# Autodesk Inventor assembly: !tower
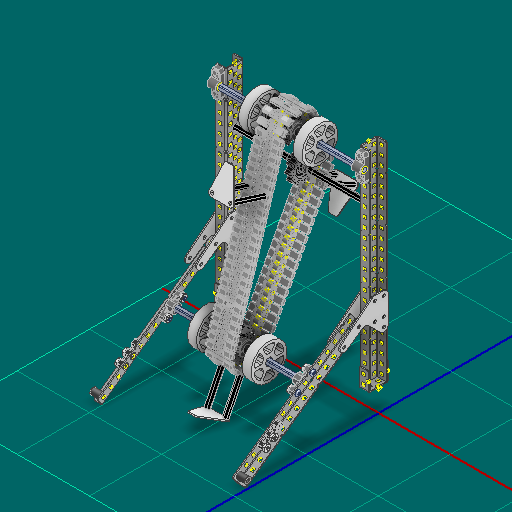
[picture p0: Inventor's stored thumbnail of the model, 512x512]
Saved by Autodesk Inventor 2025 (Build 290162000, 162)
## iProperties
Created: 2024-10-13
Part Number: !tower
Document SubType Name: Assembly
Designer: Averey Ku
Author: Averey Ku
## Documents named in this file (26)
- C:\Users\avere\vex_robotics_high_stakes\hardware\cad\bots\high_stakes_v2\tower\!tower.iam
- C:\Users\avere\vex_robotics_high_stakes\hardware\cad\bots\high_stakes_v2\tower\structure\!structure.iam
- C:\Users\avere\vex_robotics_high_stakes\hardware\cad\robpros_cad_lib\Motion\Shaft HS\Shaft HS\Shaft HS 7.5 in.ipt
- C:\Users\avere\vex_robotics_high_stakes\hardware\cad\robpros_cad_lib\Motion\Sprockets\9P Sprocket\9P 12T Sprocket, No Insert.iam
- C:\Users\avere\vex_robotics_high_stakes\hardware\cad\robpros_cad_lib\Motion\Wheels\Flex Wheels\2.000 Flex Wheel\2.000 30A .500.ipt
- C:\Users\avere\vex_robotics_high_stakes\hardware\cad\robpros_cad_lib\Motion\Shaft HS\Shaft HS\Shaft HS 8.5 in.ipt
- C:\Users\avere\vex_robotics_high_stakes\hardware\cad\bots\high_stakes_v2\tower\chain_path.ipt
- C:\Users\avere\vex_robotics_high_stakes\hardware\cad\robpros_cad_lib\Motion\Chain 9P\Tank Tread Traction Link.ipt
- C:\Users\avere\vex_robotics_high_stakes\hardware\cad\robpros_cad_lib\Motion\Chain 9P\Chain Attachment Link.ipt
- C:\Users\avere\vex_robotics_high_stakes\hardware\cad\robpros_cad_lib\Structure\Standoff\Standoff .25.ipt
- C:\Users\avere\vex_robotics_high_stakes\hardware\cad\robpros_cad_lib\Structure\Standoff\Standoff 3.00.ipt
- C:\Users\avere\vex_robotics_high_stakes\hardware\cad\robpros_cad_lib\Motion\Spacers\Spacer Nylon .375 OD\NSpacer .375 OD x .125.ipt
- C:\Users\avere\vex_robotics_high_stakes\hardware\cad\robpros_cad_lib\Motion\Spacers\Washer Steel\SWasher .375 OD x .031250.ipt
- C:\Users\avere\vex_robotics_high_stakes\hardware\cad\robpros_cad_lib\Structure\Standoff\Standoff 2.00.ipt
- C:\Users\avere\vex_robotics_high_stakes\hardware\cad\bots\high_stakes_v2\intake\custom_parts\hook_gusset.ipt
- C:\Users\avere\vex_robotics_high_stakes\hardware\cad\robpros_cad_lib\Motion\Shaft HS\HS Spacer\HSpacer .0625.ipt
- C:\Users\avere\vex_robotics_high_stakes\hardware\cad\robpros_cad_lib\Motion\Shaft HS\HS Spacer.ipt
- C:\Users\avere\vex_robotics_high_stakes\hardware\cad\robpros_cad_lib\Motion\Shaft HS\HS Spacer\HSpacer .1250.ipt
- C:\Users\avere\vex_robotics_high_stakes\hardware\cad\robpros_cad_lib\Motion\Shaft HS\HS Spacer\HSpacer .5000.ipt
- C:\Users\avere\vex_robotics_high_stakes\hardware\cad\robpros_cad_lib\Motion\Shaft HS\Low Profile HS Shaft Collar.ipt
- C:\Users\avere\vex_robotics_high_stakes\hardware\cad\robpros_cad_lib\Motion\Shaft HS\Shaft HS.ipt
- C:\Users\avere\vex_robotics_high_stakes\hardware\cad\robpros_cad_lib\Motion\Sprockets\9P Sprocket.iam
- C:\Users\avere\vex_robotics_high_stakes\hardware\cad\robpros_cad_lib\Motion\Wheels\Flex Wheels\2.000 Flex Wheel.ipt
- C:\Users\avere\vex_robotics_high_stakes\hardware\cad\robpros_cad_lib\Structure\Standoff.ipt
- C:\Users\avere\vex_robotics_high_stakes\hardware\cad\robpros_cad_lib\Motion\Spacers\Spacer Nylon .375 OD.ipt
- C:\Users\avere\vex_robotics_high_stakes\hardware\cad\robpros_cad_lib\Motion\Spacers\Washer Steel.ipt
## Components (111 placed, 18 different names)
1. !structure:1 [sub-assembly] — Insert:1, Insert:2, Insert:5, Insert:11, Insert:17
2. Shaft HS 7.5 in:1 — Insert:1
3. 9P 12T Sprocket, No Insert:2 [sub-assembly] — Insert:2, Insert:3, Insert:4, Flush:1, Flush:3, Insert:41, Insert:42
4. 2.000 30A .500:1 — Insert:3
5. 2.000 30A .500:2 — Insert:4
6. Shaft HS 8.5 in:2 — Insert:5, Mate:1
7. 9P 12T Sprocket, No Insert:3 [sub-assembly] — Flush:1, Mate:1, Insert:6, Insert:7, Flush:2, Mate:3, Insert:49, Insert:50
8. 2.000 30A .500:3 — Insert:6
9. 2.000 30A .500:4 — Insert:7
10. 9P 12T Sprocket, No Insert:4 [sub-assembly] — Flush:2
11. chain_path:1 — Flush:3, Mate:4, Angle:1
12. Chain Attachment Link:1 — Insert:9, Mate:5
13. Standoff .25:1 — Insert:10, Insert:13
14. Standoff 3.00:2 — Insert:10, Insert:11
15. NSpacer .375 OD x .125:1 — Insert:12, Insert:13
16. SWasher .375 OD x .031250:1 — Insert:12
17. Standoff .25:3
18. Standoff 3.00:4 — Insert:17
19. NSpacer .375 OD x .125:2
20. SWasher .375 OD x .031250:2
21. Standoff 2.00:7 — Mate:9
22. Standoff 2.00:8 — Insert:25
23. Chain Attachment Link:3 — Insert:24, Mate:8
24. hook_gusset:2 — Insert:25, Mate:9
25. Standoff 2.00:9
26. Standoff 2.00:10
27. Chain Attachment Link:4 — Insert:29, Mate:11
28. hook_gusset:3
29. Standoff 2.00:11
30. Standoff 2.00:12
31. Chain Attachment Link:5 — Insert:33, Mate:13
32. hook_gusset:4
33. HSpacer .0625:4 — Insert:37
34. HSpacer .1250:5 — Insert:36, Insert:37
35. HSpacer .5000:6 — Insert:35, Insert:36
36. Low Profile HS Shaft Collar:2 — Insert:35, Insert:41
37. HSpacer .0625:7
38. HSpacer .1250:8
39. HSpacer .5000:9
40. Low Profile HS Shaft Collar:3 — Insert:42
41. HSpacer .0625:10
42. HSpacer .1250:11
43. HSpacer .5000:12
44. Low Profile HS Shaft Collar:4 — Insert:50
45. HSpacer .0625:13
46. HSpacer .1250:14
47. HSpacer .5000:15
48. Low Profile HS Shaft Collar:5 — Insert:49
49. Tank Tread Traction Link:1 — Mate:3, Mate:4, Angle:1
50. Tank Tread Traction Link:2
51. Tank Tread Traction Link:3
52. Tank Tread Traction Link:4
53. Tank Tread Traction Link:5
54. Tank Tread Traction Link:6
55. Tank Tread Traction Link:7
56. Tank Tread Traction Link:8
57. Tank Tread Traction Link:9
58. Tank Tread Traction Link:10
59. Tank Tread Traction Link:11
60. Tank Tread Traction Link:12
61. Tank Tread Traction Link:13
62. Tank Tread Traction Link:14
63. Tank Tread Traction Link:15
64. Tank Tread Traction Link:16
65. Tank Tread Traction Link:17
66. Tank Tread Traction Link:18
67. Tank Tread Traction Link:19 — Insert:33, Mate:13
68. Tank Tread Traction Link:20
69. Tank Tread Traction Link:21
70. Tank Tread Traction Link:22
71. Tank Tread Traction Link:23
72. Tank Tread Traction Link:24
73. Tank Tread Traction Link:25
74. Tank Tread Traction Link:26
75. Tank Tread Traction Link:27
76. Tank Tread Traction Link:28
77. Tank Tread Traction Link:29
78. Tank Tread Traction Link:30
79. Tank Tread Traction Link:31
80. Tank Tread Traction Link:32
81. Tank Tread Traction Link:33
82. Tank Tread Traction Link:34
83. Tank Tread Traction Link:35
84. Tank Tread Traction Link:36
85. Tank Tread Traction Link:37
86. Tank Tread Traction Link:38
87. Tank Tread Traction Link:39
88. Tank Tread Traction Link:40 — Insert:29, Mate:11
89. Tank Tread Traction Link:41
90. Tank Tread Traction Link:42
91. Tank Tread Traction Link:43
92. Tank Tread Traction Link:44
93. Tank Tread Traction Link:45
94. Tank Tread Traction Link:46
95. Tank Tread Traction Link:47
96. Tank Tread Traction Link:48
97. Tank Tread Traction Link:49
98. Tank Tread Traction Link:50
99. Tank Tread Traction Link:51
100. Tank Tread Traction Link:52
101. Tank Tread Traction Link:53 — Insert:9, Mate:5
102. Tank Tread Traction Link:54
103. Tank Tread Traction Link:55
104. Tank Tread Traction Link:56
105. Tank Tread Traction Link:57
106. Tank Tread Traction Link:58
107. Tank Tread Traction Link:59
108. Tank Tread Traction Link:60
109. Tank Tread Traction Link:61 — Insert:24, Mate:8
110. Tank Tread Traction Link:62
111. Tank Tread Traction Link:63
## Component patterns: (63 elements, first: Tank Tread Traction Link:1)
## Relationships (58: Insert 44, Mate 10, Flush 3, Angle 1)
- Insert:1: !structure:1 ↔ Shaft HS 7.5 in:1
- Insert:2 (87.9094 mm): !structure:1 ↔ 9P 12T Sprocket, No Insert:2
- Insert:3 (25.4 mm): 9P 12T Sprocket, No Insert:2 ↔ 2.000 30A .500:1
- Insert:4 (25.4 mm): 9P 12T Sprocket, No Insert:2 ↔ 2.000 30A .500:2
- Insert:5: !structure:1 ↔ Shaft HS 8.5 in:2
- Flush:1: 9P 12T Sprocket, No Insert:2 ↔ 9P 12T Sprocket, No Insert:3
- Mate:1: Shaft HS 8.5 in:2 ↔ 9P 12T Sprocket, No Insert:3
- Insert:6 (25.4 mm): 9P 12T Sprocket, No Insert:3 ↔ 2.000 30A .500:3
- Insert:7 (25.4 mm): 9P 12T Sprocket, No Insert:3 ↔ 2.000 30A .500:4
- Flush:2: 9P 12T Sprocket, No Insert:3 ↔ 9P 12T Sprocket, No Insert:4
- Flush:3: 9P 12T Sprocket, No Insert:2 ↔ chain_path:1
- Mate:3: 9P 12T Sprocket, No Insert:3 ↔ Tank Tread Traction Link:1
- Mate:4: chain_path:1 ↔ Tank Tread Traction Link:1
- Angle:1 (-90 deg): chain_path:1 ↔ Tank Tread Traction Link:1
- Insert:9: Chain Attachment Link:1 ↔ Tank Tread Traction Link:53
- Mate:5: Chain Attachment Link:1 ↔ Tank Tread Traction Link:53
- Insert:10: Standoff .25:1 ↔ Standoff 3.00:2
- Insert:11: !structure:1 ↔ Standoff 3.00:2
- Insert:12: NSpacer .375 OD x .125:1 ↔ SWasher .375 OD x .031250:1
- Insert:13: Standoff .25:1 ↔ NSpacer .375 OD x .125:1
- [Insert]: Standoff .25:3 ↔ Standoff 3.00:4
- [Insert]: NSpacer .375 OD x .125:2 ↔ SWasher .375 OD x .031250:2
- [Insert]: Standoff .25:3 ↔ NSpacer .375 OD x .125:2
- Insert:17: !structure:1 ↔ Standoff 3.00:4
- [Insert]: Standoff 2.00:8 ↔ Chain Attachment Link:3
- [Insert]: Standoff 2.00:7 ↔ Chain Attachment Link:3
- Insert:24: Chain Attachment Link:3 ↔ Tank Tread Traction Link:61
- Mate:8: Chain Attachment Link:3 ↔ Tank Tread Traction Link:61
- Insert:25: Standoff 2.00:8 ↔ hook_gusset:2
- Mate:9: Standoff 2.00:7 ↔ hook_gusset:2
- [Insert]: Standoff 2.00:10 ↔ Chain Attachment Link:4
- [Insert]: Standoff 2.00:9 ↔ Chain Attachment Link:4
- [Insert]: Standoff 2.00:10 ↔ hook_gusset:3
- [Mate]: Standoff 2.00:9 ↔ hook_gusset:3
- Insert:29: Chain Attachment Link:4 ↔ Tank Tread Traction Link:40
- Mate:11: Chain Attachment Link:4 ↔ Tank Tread Traction Link:40
- [Insert]: Standoff 2.00:12 ↔ Chain Attachment Link:5
- [Insert]: Standoff 2.00:11 ↔ Chain Attachment Link:5
- [Insert]: Standoff 2.00:12 ↔ hook_gusset:4
- [Mate]: Standoff 2.00:11 ↔ hook_gusset:4
- Insert:33: Chain Attachment Link:5 ↔ Tank Tread Traction Link:19
- Mate:13: Chain Attachment Link:5 ↔ Tank Tread Traction Link:19
- Insert:35: HSpacer .5000:6 ↔ Low Profile HS Shaft Collar:2
- Insert:36: HSpacer .1250:5 ↔ HSpacer .5000:6
- Insert:37: HSpacer .0625:4 ↔ HSpacer .1250:5
- [Insert]: HSpacer .5000:9 ↔ Low Profile HS Shaft Collar:3
- [Insert]: HSpacer .1250:8 ↔ HSpacer .5000:9
- [Insert]: HSpacer .0625:7 ↔ HSpacer .1250:8
- Insert:41: 9P 12T Sprocket, No Insert:2 ↔ Low Profile HS Shaft Collar:2
- Insert:42: 9P 12T Sprocket, No Insert:2 ↔ Low Profile HS Shaft Collar:3
- [Insert]: HSpacer .5000:12 ↔ Low Profile HS Shaft Collar:4
- [Insert]: HSpacer .1250:11 ↔ HSpacer .5000:12
- [Insert]: HSpacer .0625:10 ↔ HSpacer .1250:11
- [Insert]: HSpacer .5000:15 ↔ Low Profile HS Shaft Collar:5
- [Insert]: HSpacer .1250:14 ↔ HSpacer .5000:15
- [Insert]: HSpacer .0625:13 ↔ HSpacer .1250:14
- Insert:49: 9P 12T Sprocket, No Insert:3 ↔ Low Profile HS Shaft Collar:5
- Insert:50: 9P 12T Sprocket, No Insert:3 ↔ Low Profile HS Shaft Collar:4
## Named parameters: d31_d27 = 0 mm, d32_d29 = 0 mm, d33_d30 = 0 mm, d45_d35 = 0 mm, d46_d36 = 0 mm, d51_d45_d35 = 0 mm, d52_d46_d36 = 0 mm, d53_d49 = 0 mm, d54_d50 = 0 mm, d57_d51_d45_d35 = 0 mm, d58_d52_d46_d36 = 0 mm, d59_d53_d49 = 0 mm, d60_d54_d50 = 0 mm, d67_d64 = 0 mm, d68_d65 = 0 mm, d69_d66 = 0 mm, d72_d64 = 0 mm, d73_d65 = 0 mm, d74_d66 = 0 mm, d75_d64 = 0 mm, d76_d65 = 0 mm, d77_d66 = 0 mm
